# Autodesk Inventor assembly: Servo Arm
Saved by Autodesk Inventor 2014 SP1 (Build 180222100, 222)
## iProperties
Created: 2014-04-09
Part Number: Servo Arm
Document SubType Name: Assembly
Designer: tom
Author: tom
## Documents named in this file (4)
- C:\Users\tom\Documents\GitHub\Delta_Robots\Delatabot - Small Model\Inventor\Deltabot - Small Model ver12\Servo Arm.iam
- C:\Users\tom\Documents\GitHub\Delta_Robots\Delatabot - Small Model\Inventor\Deltabot - Small Model ver12\Servo Hub.ipt
- C:\Users\tom\Documents\GitHub\Delta_Robots\Delatabot - Small Model\Inventor\Deltabot - Small Model ver12\Linkage Mount.ipt
- C:\Users\tom\Documents\GitHub\Delta_Robots\Delatabot - Small Model\Inventor\Deltabot - Small Model ver12\Bearing.ipt
## Components (4 placed, 3 different names)
1. Servo Hub:1
2. Linkage Mount:1
3. Bearing:1
4. Bearing:2
## Relationships (2: RevoluteJoint 2)
- [RevoluteJoint]: Linkage Mount:1 ↔ Bearing:1
- [RevoluteJoint]: Linkage Mount:1 ↔ Bearing:2
